# Autodesk Inventor assembly: BodyAssembly
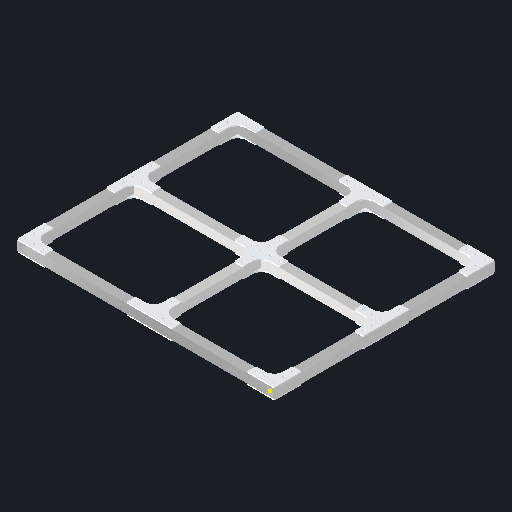
[picture p0: Inventor's stored thumbnail of the model, 512x512]
Saved by Autodesk Inventor 2024 (Build 280153000, 153)
## iProperties
Created: 2023-09-27
Part Number: BodyAssembly
Document SubType Name: Assembly
Designer: Megan
Author: Megan
## Documents named in this file (8)
- C:\Users\bugme\OneDrive - The Pennsylvania State University\Documents\GitHub\BehrendURCMechanical\CAD\Chassis V3\Body\BodyAssembly.iam
- C:\Users\bugme\OneDrive - The Pennsylvania State University\Documents\GitHub\BehrendURCMechanical\CAD\Chassis V3\Body\60cmTube.ipt
- C:\Users\bugme\OneDrive - The Pennsylvania State University\Documents\GitHub\BehrendURCMechanical\CAD\Chassis V3\Body\64cmTube.ipt
- C:\Users\bugme\OneDrive - The Pennsylvania State University\Documents\GitHub\BehrendURCMechanical\CAD\Chassis V3\Body\44.92cmTube.ipt
- C:\Users\bugme\OneDrive - The Pennsylvania State University\Documents\GitHub\BehrendURCMechanical\CAD\Chassis V3\Body\54.92Shaft.ipt
- C:\Users\bugme\OneDrive - The Pennsylvania State University\Documents\GitHub\BehrendURCMechanical\CAD\Chassis V3\Body\am-3860 90 Gusset REV2.ipt
- C:\Users\bugme\OneDrive - The Pennsylvania State University\Documents\GitHub\BehrendURCMechanical\CAD\Chassis V3\Body\am-4159 1IN Quad Gusset.ipt
- C:\Users\bugme\OneDrive - The Pennsylvania State University\Documents\GitHub\BehrendURCMechanical\CAD\Chassis V3\Body\am-4158 1IN Tee Gusset.ipt
## Components (25 placed, 8 different names)
1. 60cmTube:1 — Mate:1, Flush:1, Flush:2, Mate:2, Flush:3, Flush:4, Mate:5, Mate:6, Flush:9, Flush:16, Mate:12, Flush:18, Mate:13, Flush:21, Flush:22, Mate:14, Mate:23, Flush:41, Mate:24, Flush:43
2. 60cmTube:2 — Mate:3, Flush:5, Flush:6, Flush:10, Mate:9, Flush:12, Mate:10, Flush:15, Mate:15, Flush:25, Mate:16, Flush:27, Mate:19, Flush:32, Mate:20, Flush:34
3. 64cmTube:1 — Mate:1, Flush:1, Flush:2, Mate:3, Flush:5, Flush:6, Flush:8, Flush:20, Flush:23, Flush:24, Flush:26, Mate:25, Flush:44, Flush:47
4. 64cmTube:2 — Mate:2, Flush:3, Flush:4, Mate:4, Mate:7, Flush:13, Flush:14, Mate:11, Flush:17, Flush:19, Mate:21, Flush:37, Mate:22, Flush:38
5. 54.92cmTube:1 — Flush:7, Mate:4, Flush:8, Mate:5, Mate:8, Mate:17, Flush:29, Mate:18, Flush:30, Flush:36, Flush:39, Flush:45, Mate:26, Flush:46
6. 30.73cmTube — Mate:6, Flush:9, Mate:7, Flush:11, Flush:28, Flush:31, Flush:40, Flush:42
7. 54.92Shaft:2 — Flush:10, Mate:8, Flush:11, Flush:33, Flush:35
8. am-3860 90 Gusset REV2:1 — Mate:9, Flush:12, Flush:13
9. am-3860 90 Gusset REV2:2 — Mate:10, Flush:14, Flush:15
10. am-3860 90 Gusset REV2:3 — Mate:11, Flush:16, Flush:17
11. am-3860 90 Gusset REV2:4 — Mate:12, Flush:18, Flush:19
12. am-3860 90 Gusset REV2:5 — Mate:15, Flush:24, Flush:25
13. am-3860 90 Gusset REV2:6 — Mate:16, Flush:26, Flush:27
14. am-3860 90 Gusset REV2:7 — Mate:13, Flush:20, Flush:21
15. am-3860 90 Gusset REV2:8 — Flush:22, Flush:23, Mate:14
16. am-4159 1IN Quad Gusset:1 — Mate:17, Flush:28, Flush:29
17. am-4159 1IN Quad Gusset:2 — Mate:18, Flush:30, Flush:31
18. am-4158 1IN Tee Gusset:1 — Mate:19, Flush:32, Flush:33
19. am-4158 1IN Tee Gusset:2 — Mate:20, Flush:34, Flush:35
20. am-4158 1IN Tee Gusset:3 — Mate:21, Flush:36, Flush:37
21. am-4158 1IN Tee Gusset:4 — Mate:22, Flush:38, Flush:39
22. am-4158 1IN Tee Gusset:5 — Mate:23, Flush:40, Flush:41
23. am-4158 1IN Tee Gusset:6 — Mate:24, Flush:42, Flush:43
24. am-4158 1IN Tee Gusset:7 — Mate:25, Flush:44, Flush:45
25. am-4158 1IN Tee Gusset:8 — Mate:26, Flush:46, Flush:47
## Relationships (73: Flush 47, Mate 26)
- Mate:1: 60cmTube:1 ↔ 64cmTube:1
- Flush:1: 60cmTube:1 ↔ 64cmTube:1
- Flush:2: 60cmTube:1 ↔ 64cmTube:1
- Mate:2: 60cmTube:1 ↔ 64cmTube:2
- Flush:3: 60cmTube:1 ↔ 64cmTube:2
- Flush:4: 60cmTube:1 ↔ 64cmTube:2
- Mate:3: 60cmTube:2 ↔ 64cmTube:1
- Flush:5: 60cmTube:2 ↔ 64cmTube:1
- Flush:6: 60cmTube:2 ↔ 64cmTube:1
- Flush:7: 54.92cmTube:1
- Mate:4: 64cmTube:2 ↔ 54.92cmTube:1
- Flush:8: 64cmTube:1 ↔ 54.92cmTube:1
- Mate:5 (307.3 mm): 60cmTube:1 ↔ 54.92cmTube:1
- Mate:6: 60cmTube:1 ↔ 30.73cmTube
- Flush:9: 60cmTube:1 ↔ 30.73cmTube
- Mate:7 (261.9 mm): 64cmTube:2 ↔ 30.73cmTube
- Flush:10: 60cmTube:2 ↔ 54.92Shaft:2
- Mate:8: 54.92cmTube:1 ↔ 54.92Shaft:2
- Flush:11: 30.73cmTube ↔ 54.92Shaft:2
- Mate:9: 60cmTube:2 ↔ am-3860 90 Gusset REV2:1
- Flush:12: 60cmTube:2 ↔ am-3860 90 Gusset REV2:1
- Flush:13: 64cmTube:2 ↔ am-3860 90 Gusset REV2:1
- Mate:10: 60cmTube:2 ↔ am-3860 90 Gusset REV2:2
- Flush:14: 64cmTube:2 ↔ am-3860 90 Gusset REV2:2
- Flush:15: 60cmTube:2 ↔ am-3860 90 Gusset REV2:2
- Mate:11: 64cmTube:2 ↔ am-3860 90 Gusset REV2:3
- Flush:16: 60cmTube:1 ↔ am-3860 90 Gusset REV2:3
- Flush:17: 64cmTube:2 ↔ am-3860 90 Gusset REV2:3
- Mate:12: 60cmTube:1 ↔ am-3860 90 Gusset REV2:4
- Flush:18: 60cmTube:1 ↔ am-3860 90 Gusset REV2:4
- Flush:19: 64cmTube:2 ↔ am-3860 90 Gusset REV2:4
- Mate:13: 60cmTube:1 ↔ am-3860 90 Gusset REV2:7
- Flush:20: 64cmTube:1 ↔ am-3860 90 Gusset REV2:7
- Flush:21: 60cmTube:1 ↔ am-3860 90 Gusset REV2:7
- Flush:22: 60cmTube:1 ↔ am-3860 90 Gusset REV2:8
- Flush:23: 64cmTube:1 ↔ am-3860 90 Gusset REV2:8
- Mate:14: 60cmTube:1 ↔ am-3860 90 Gusset REV2:8
- Mate:15: 60cmTube:2 ↔ am-3860 90 Gusset REV2:5
- Flush:24: 64cmTube:1 ↔ am-3860 90 Gusset REV2:5
- Flush:25: 60cmTube:2 ↔ am-3860 90 Gusset REV2:5
- Mate:16: 60cmTube:2 ↔ am-3860 90 Gusset REV2:6
- Flush:26: 64cmTube:1 ↔ am-3860 90 Gusset REV2:6
- Flush:27: 60cmTube:2 ↔ am-3860 90 Gusset REV2:6
- Mate:17: 54.92cmTube:1 ↔ am-4159 1IN Quad Gusset:1
- Flush:28: 30.73cmTube ↔ am-4159 1IN Quad Gusset:1
- Flush:29: 54.92cmTube:1 ↔ am-4159 1IN Quad Gusset:1
- Mate:18: 54.92cmTube:1 ↔ am-4159 1IN Quad Gusset:2
- Flush:30: 54.92cmTube:1 ↔ am-4159 1IN Quad Gusset:2
- Flush:31: 30.73cmTube ↔ am-4159 1IN Quad Gusset:2
- Mate:19: 60cmTube:2 ↔ am-4158 1IN Tee Gusset:1
- Flush:32: 60cmTube:2 ↔ am-4158 1IN Tee Gusset:1
- Flush:33: 54.92Shaft:2 ↔ am-4158 1IN Tee Gusset:1
- Mate:20: 60cmTube:2 ↔ am-4158 1IN Tee Gusset:2
- Flush:34: 60cmTube:2 ↔ am-4158 1IN Tee Gusset:2
- Flush:35: 54.92Shaft:2 ↔ am-4158 1IN Tee Gusset:2
- Mate:21: 64cmTube:2 ↔ am-4158 1IN Tee Gusset:3
- Flush:36: 54.92cmTube:1 ↔ am-4158 1IN Tee Gusset:3
- Flush:37: 64cmTube:2 ↔ am-4158 1IN Tee Gusset:3
- Mate:22: 64cmTube:2 ↔ am-4158 1IN Tee Gusset:4
- Flush:38: 64cmTube:2 ↔ am-4158 1IN Tee Gusset:4
- Flush:39: 54.92cmTube:1 ↔ am-4158 1IN Tee Gusset:4
- Mate:23: 60cmTube:1 ↔ am-4158 1IN Tee Gusset:5
- Flush:40: 30.73cmTube ↔ am-4158 1IN Tee Gusset:5
- Flush:41: 60cmTube:1 ↔ am-4158 1IN Tee Gusset:5
- Mate:24: 60cmTube:1 ↔ am-4158 1IN Tee Gusset:6
- Flush:42: 30.73cmTube ↔ am-4158 1IN Tee Gusset:6
- Flush:43: 60cmTube:1 ↔ am-4158 1IN Tee Gusset:6
- Mate:25: 64cmTube:1 ↔ am-4158 1IN Tee Gusset:7
- Flush:44: 64cmTube:1 ↔ am-4158 1IN Tee Gusset:7
- Flush:45: 54.92cmTube:1 ↔ am-4158 1IN Tee Gusset:7
- Mate:26: 54.92cmTube:1 ↔ am-4158 1IN Tee Gusset:8
- Flush:46: 54.92cmTube:1 ↔ am-4158 1IN Tee Gusset:8
- Flush:47: 64cmTube:1 ↔ am-4158 1IN Tee Gusset:8
